# Autodesk Inventor assembly: ASSEMBLY_piston
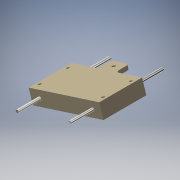
[picture p0: Inventor's stored thumbnail of the model, 180x180]
Saved by Autodesk Inventor 2018 (Build 220112000, 112)
## iProperties
Created: 2026-05-31
Part Number: ASSEMBLY_piston
Document SubType Name: Assembly
Designer: neo
Author: neo
## Documents named in this file (4)
- C:\Users\neo\Documents\neoatlantis-shared\projects\kreion\design2\ASSEMBLY_piston.iam
- C:\Users\neo\Documents\neoatlantis-shared\projects\kreion\design2\PRING_piston_case_half.ipt
- C:\Users\neo\Documents\neoatlantis-shared\projects\kreion\design2\HELP_MAGNET_D10x40.ipt
- C:\Users\neo\Documents\neoatlantis-shared\projects\kreion\design2\HELP_ROD_D3x100.ipt
## Components (5 placed, 3 different names)
1. PRING_piston_case_half:1 — Tangent:1, Tangent:2, Mate:1, Mate:2, Tangent:3, Tangent:4, Tangent:5, Tangent:7, Tangent:8
2. PRING_piston_case_half:2 — Mate:2, Tangent:3, Tangent:4, Tangent:6
3. HELP_MAGNET_D10x40:1 — Tangent:1, Tangent:2, Mate:1
4. HELP_ROD_D3x100:1 — Tangent:5, Tangent:6, Flush:1
5. HELP_ROD_D3x100:2 — Tangent:7, Tangent:8, Flush:1
## Relationships (11: Tangent 8, Mate 2, Flush 1)
- Tangent:1: PRING_piston_case_half:1 ↔ HELP_MAGNET_D10x40:1
- Tangent:2: PRING_piston_case_half:1 ↔ HELP_MAGNET_D10x40:1
- Mate:1: PRING_piston_case_half:1 ↔ HELP_MAGNET_D10x40:1
- Mate:2: PRING_piston_case_half:1 ↔ PRING_piston_case_half:2
- Tangent:3: PRING_piston_case_half:1 ↔ PRING_piston_case_half:2
- Tangent:4: PRING_piston_case_half:1 ↔ PRING_piston_case_half:2
- Tangent:5: PRING_piston_case_half:1 ↔ HELP_ROD_D3x100:1
- Tangent:6: PRING_piston_case_half:2 ↔ HELP_ROD_D3x100:1
- Tangent:7: PRING_piston_case_half:1 ↔ HELP_ROD_D3x100:2
- Tangent:8: PRING_piston_case_half:1 ↔ HELP_ROD_D3x100:2
- Flush:1: HELP_ROD_D3x100:1 ↔ HELP_ROD_D3x100:2
